# Autodesk Inventor assembly: ASY ДМФ 0100 Барабан v2.1
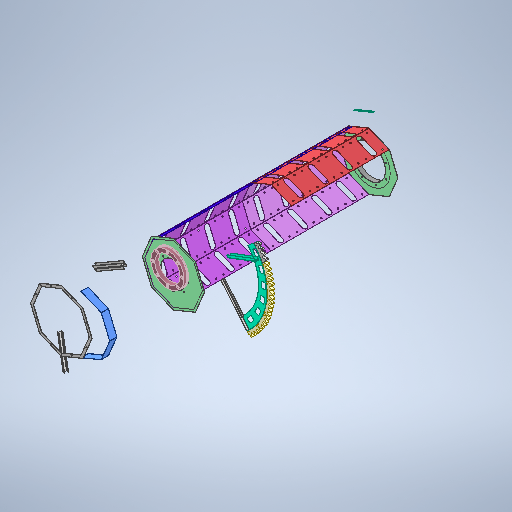
[picture p0: Inventor's stored thumbnail of the model, 512x512]
Saved by Autodesk Inventor 2026 (Build 300175000, 175)
## iProperties
Created: 2024-04-28
Part Number: ASY ДМФ 0100 Барабан v2.1
Document SubType Name: Assembly
Designer: pokla
Author: pokla
## Documents named in this file (25)
- C:\Users\pokla\Documents\Inventor\ДФО\ДМФ\DMF-Disk-Micro-Filter\Барабан v2.1\ASY ДМФ 0100 Барабан v2.1.iam
- C:\Users\pokla\Documents\Inventor\ДФО\ДМФ\DMF-Disk-Micro-Filter\Барабан v2.1\DMF 01 21 Барабан торец НОС v2.1.ipt
- C:\Users\pokla\Documents\Inventor\ДФО\ДМФ\DMF-Disk-Micro-Filter\Барабан v2.1\DMF 01 13 Барабан Лист лев брт v2.1.ipt
- C:\Users\pokla\Documents\Inventor\ДФО\ДМФ\DMF-Disk-Micro-Filter\Барабан v2.1\DMF 01 14 Барабан Лист прав брт v2.1.ipt
- C:\Users\pokla\Documents\Inventor\ДФО\ДМФ\DMF-Disk-Micro-Filter\Барабан v2.1\DMF 01 31 Барабан Опорное кольцо НОС v2.1.ipt
- C:\Users\pokla\Documents\Inventor\ДФО\ДМФ\DMF-Disk-Micro-Filter\Барабан v2.1\DMF 01 17 опора крышки v2.1.ipt
- C:\Users\pokla\Documents\Inventor\ДФО\ДМФ\DMF-Disk-Micro-Filter\Барабан v2.1\DMF 000 размеры v2.1.ipt
- C:\Users\pokla\Documents\Inventor\ДФО\ДМФ\DMF-Disk-Micro-Filter\Барабан v2.1\DMF 01 12 Барабан усилитель v2.1.ipt
- C:\Users\pokla\Documents\Inventor\ДФО\ДМФ\DMF-Disk-Micro-Filter\Барабан v2.1\ASY DMF 010 cap v2.1.iam
- C:\Users\pokla\Documents\Inventor\ДФО\ДМФ\DMF-Disk-Micro-Filter\Барабан v2.1\DMF 01 32 Барабан Опорное кольцо КОРМА v2.1.ipt
- C:\Users\pokla\Documents\Inventor\ДФО\ДМФ\DMF-Disk-Micro-Filter\Барабан v2.1\DMF 01 22 Барабан торец КОРМА v2.1.ipt
- C:\Users\pokla\Documents\Inventor\ДФО\ДМФ\DMF-Disk-Micro-Filter\Барабан v2.1\ASY DMF filter package v2.1.iam
- C:\Users\pokla\Documents\Inventor\ДФО\ДМФ\DMF-Disk-Micro-Filter\Барабан v2.1\DMF 01 21 cylinder butt end nose.ipt
- C:\Users\pokla\Documents\Inventor\ДФО\ДМФ\DMF-Disk-Micro-Filter\Барабан v2.1\DMF 2.1 01 43 Gear rim 3.ipt
- C:\Users\pokla\Documents\Inventor\ДФО\ДМФ\DMF-Disk-Micro-Filter\Барабан v2.1\DMF 2.1 01 44 Gear rim 4.ipt
- C:\Users\pokla\Documents\Inventor\ДФО\ДМФ\DMF-Disk-Micro-Filter\Барабан v2.1\DMF 2.1 01 45 Gear ring 5.ipt
- C:\Users\pokla\Documents\Inventor\ДФО\ДМФ\DMF-Disk-Micro-Filter\Барабан v2.1\DMF 2.1 01 46 Gear axis wheel 6.ipt
- C:\Users\pokla\Documents\Inventor\ДФО\ДМФ\DMF-Disk-Micro-Filter\Барабан v2.1\DMF 01 13 Барабан усилитель v2.1.ipt
- C:\Users\pokla\Documents\Inventor\ДФО\ДМФ\DMF-Disk-Micro-Filter\шестерни 06.09.2025\DMF sector big gear 2.1.ipt
- C:\Users\pokla\Documents\Inventor\ДФО\ДМФ\DMF-Disk-Micro-Filter\Барабан v2.1\DMF 01 15 drum sheet 1.ipt
- C:\Users\pokla\Documents\Inventor\ДФО\ДМФ\DMF-Disk-Micro-Filter\ДМФ 01 12 Барабан усилитель.ipt
- C:\Users\pokla\Documents\Inventor\ДФО\ДМФ\DMF-Disk-Micro-Filter\ДМФ 01 15 Барабан усилитель борта.ipt
- C:\Users\pokla\Documents\Inventor\ДФО\ДМФ\DMF-Disk-Micro-Filter\Барабан v2.1\DMF 2.1 Пластина паза маленькая.ipt
- C:\Users\pokla\Documents\Inventor\ДФО\ДМФ\DMF-Disk-Micro-Filter\Барабан v2.1\DMF 2.1 Пластина паза большая.ipt
- C:\Users\pokla\Documents\Inventor\ДФО\ДМФ\DMF-Disk-Micro-Filter\Барабан v2.1\DMF 01 11 cylinder sheet cap v2.1.ipt
## Components (43 placed, 30 different names)
1. DMF 000 размеры v2.1.ipt:1
2. DMF 01 21 Барабан торец НОС v2.1.ipt:1 — Жесткий:101, Совмещение:49
3. DMF 01 31 Барабан Опорное кольцо НОС v2.1.ipt:1
4. DMF 01 32 Барабан Опорное кольцо КОРМА v2.1.ipt:1 — Жесткий:20
5. DMF 01 22 Барабан торец КОРМА v2.1.ipt:1 — Жесткий:20, Жесткий:51, Жесткий:53, Совмещение:37, Жесткий:97, Совмещение:46
6. DMF 01 13 Барабан Лист лев брт v2.1.ipt:1 — Жесткий:51, Жесткий:98
7. DMF 01 14 Барабан Лист прав брт v2.1.ipt:1 — Жесткий:53
8. DMF 01 17 опора крышки v2.1.ipt:1 — Совмещение:37, Совмещение:46, Совмещение:47, Совмещение:48, Жесткий:112
9. DMF 01 11 cylinder sheet cap v2.1.ipt:1 — Совмещение:47, Жесткий:100
10. ASY DMF 010 cap v2.1.iam:1 [sub-assembly]
11. DMF 01 21 cylinder butt end nose.ipt:1
12. DMF 2.1 01 45 Gear ring 5.ipt:1
13. DMF 2.1 01 46 Gear axis wheel 6.ipt:1
14. DMF 2.1 01 44 Gear rim 4.ipt:1 — Жесткий:102, Жесткий:110
15. DMF 2.1 01 43 Gear rim 3.ipt:2 — Жесткий:102, Жесткий:103, Жесткий:109
16. DMF 01 15 drum sheet 1.ipt:1
17. ДМФ 01 12 Барабан усилитель.ipt:2 — Жесткий:56, Жесткий:57, Жесткий:89
18. ДМФ 01 15 Барабан усилитель борта.ipt:3 — Жесткий:56
19. ДМФ 01 15 Барабан усилитель борта.ipt:4 — Жесткий:57
20. ДМФ 01 12 Барабан усилитель:3 — Жесткий:89
21. ДМФ 01 15 Барабан усилитель борта:5
22. ДМФ 01 15 Барабан усилитель борта:6
23. DMF 01 12 Барабан усилитель v2.1.ipt:1 — Жесткий:82
24. DMF 01 13 Барабан усилитель v2.1.ipt:1 — Жесткий:82
25. DMF 01 12 Барабан усилитель v2.1.ipt:2
26. DMF 01 13 Барабан усилитель v2.1.ipt:2 — Жесткий:103
27. DMF 2.1 Пластина паза маленькая.ipt:1
28. DMF 2.1 Пластина паза большая:1 — Жесткий:110, Совмещение:49
29. ASY DMF filter package v2.1.iam:1 [sub-assembly]
30. DMF sector big gear 2.1.ipt:1 — Жесткий:104, Жесткий:109
31. ASY DMF filter package v2.1:2 [sub-assembly]
32. ASY DMF filter package v2.1:3 [sub-assembly]
33. ASY DMF filter package v2.1:4 [sub-assembly]
34. DMF 01 13 Барабан Лист лев брт v2.1:2 — Жесткий:97, Жесткий:99, Совмещение:48
35. DMF 01 13 Барабан Лист лев брт v2.1:3 — Жесткий:98
36. DMF 01 13 Барабан Лист лев брт v2.1:4 — Жесткий:99, Жесткий:101
37. DMF sector big gear 2.1:2 — Жесткий:104, Жесткий:105
38. DMF sector big gear 2.1:3 — Жесткий:105, Жесткий:106
39. DMF sector big gear 2.1:4 — Жесткий:106, Жесткий:107
40. DMF sector big gear 2.1:5 — Жесткий:107, Жесткий:108
41. DMF sector big gear 2.1:6 — Жесткий:108
42. ASY DMF filter package v2.1:5 [sub-assembly] — Жесткий:100
43. DMF 01 17 опора крышки v2.1:4 — Жесткий:112
## Relationships (34: WeldJoint 26, Mate 6, Flush 2)
- Жесткий:20 [WeldJoint]: DMF 01 32 Барабан Опорное кольцо КОРМА v2.1.ipt:1 ↔ DMF 01 22 Барабан торец КОРМА v2.1.ipt:1
- Жесткий:51 [WeldJoint]: DMF 01 22 Барабан торец КОРМА v2.1.ipt:1 ↔ DMF 01 13 Барабан Лист лев брт v2.1.ipt:1
- Жесткий:53 [WeldJoint]: DMF 01 22 Барабан торец КОРМА v2.1.ipt:1 ↔ DMF 01 14 Барабан Лист прав брт v2.1.ipt:1
- Совмещение:37 [Mate]: DMF 01 22 Барабан торец КОРМА v2.1.ipt:1 ↔ DMF 01 17 опора крышки v2.1.ipt:1
- Жесткий:56 [WeldJoint]: ДМФ 01 12 Барабан усилитель.ipt:2 ↔ ДМФ 01 15 Барабан усилитель борта.ipt:3
- Жесткий:57 [WeldJoint]: ДМФ 01 12 Барабан усилитель.ipt:2 ↔ ДМФ 01 15 Барабан усилитель борта.ipt:4
- [Mate]: DMF 01 22 Барабан торец КОРМА v2.1.ipt:1 ↔ DMF 01 11 cylinder sheet cap v2.1.ipt:1
- [Flush]: DMF 01 22 Барабан торец КОРМА v2.1.ipt:1 ↔ DMF 01 11 cylinder sheet cap v2.1.ipt:1
- [Flush]: DMF 01 22 Барабан торец КОРМА v2.1.ipt:1 ↔ DMF 01 11 cylinder sheet cap v2.1.ipt:1
- Жесткий:82 [WeldJoint]: DMF 01 12 Барабан усилитель v2.1.ipt:1 ↔ DMF 01 13 Барабан усилитель v2.1.ipt:1
- [WeldJoint]: ДМФ 01 12 Барабан усилитель:3 ↔ ДМФ 01 15 Барабан усилитель борта:5
- [WeldJoint]: ДМФ 01 12 Барабан усилитель:3 ↔ ДМФ 01 15 Барабан усилитель борта:6
- Жесткий:89 [WeldJoint]: ДМФ 01 12 Барабан усилитель.ipt:2 ↔ ДМФ 01 12 Барабан усилитель:3
- [WeldJoint]: DMF 01 11 cylinder sheet cap v2.1.ipt:1 ↔ ASY DMF filter package v2.1.iam:1
- [WeldJoint]: DMF 01 11 cylinder sheet cap v2.1.ipt:1 ↔ ASY DMF filter package v2.1:2
- Жесткий:97 [WeldJoint]: DMF 01 22 Барабан торец КОРМА v2.1.ipt:1 ↔ DMF 01 13 Барабан Лист лев брт v2.1:2
- Жесткий:98 [WeldJoint]: DMF 01 13 Барабан Лист лев брт v2.1.ipt:1 ↔ DMF 01 13 Барабан Лист лев брт v2.1:3
- Жесткий:99 [WeldJoint]: DMF 01 13 Барабан Лист лев брт v2.1:2 ↔ DMF 01 13 Барабан Лист лев брт v2.1:4
- Совмещение:46 [Mate]: DMF 01 22 Барабан торец КОРМА v2.1.ipt:1 ↔ DMF 01 17 опора крышки v2.1.ipt:1
- Совмещение:47 [Mate]: DMF 01 17 опора крышки v2.1.ipt:1 ↔ DMF 01 11 cylinder sheet cap v2.1.ipt:1
- Совмещение:48 [Mate]: DMF 01 17 опора крышки v2.1.ipt:1 ↔ DMF 01 13 Барабан Лист лев брт v2.1:2
- Жесткий:100 [WeldJoint]: DMF 01 11 cylinder sheet cap v2.1.ipt:1 ↔ ASY DMF filter package v2.1:5
- Жесткий:101 [WeldJoint]: DMF 01 21 Барабан торец НОС v2.1.ipt:1 ↔ DMF 01 13 Барабан Лист лев брт v2.1:4
- Жесткий:102 [WeldJoint]: DMF 2.1 01 44 Gear rim 4.ipt:1 ↔ DMF 2.1 01 43 Gear rim 3.ipt:2
- Жесткий:103 [WeldJoint]: DMF 2.1 01 43 Gear rim 3.ipt:2 ↔ DMF 01 13 Барабан усилитель v2.1.ipt:2
- Жесткий:104 [WeldJoint]: DMF sector big gear 2.1.ipt:1 ↔ DMF sector big gear 2.1:2
- Жесткий:105 [WeldJoint]: DMF sector big gear 2.1:2 ↔ DMF sector big gear 2.1:3
- Жесткий:106 [WeldJoint]: DMF sector big gear 2.1:3 ↔ DMF sector big gear 2.1:4
- Жесткий:107 [WeldJoint]: DMF sector big gear 2.1:4 ↔ DMF sector big gear 2.1:5
- Жесткий:108 [WeldJoint]: DMF sector big gear 2.1:5 ↔ DMF sector big gear 2.1:6
- Жесткий:109 [WeldJoint]: DMF 2.1 01 43 Gear rim 3.ipt:2 ↔ DMF sector big gear 2.1.ipt:1
- Жесткий:110 [WeldJoint]: DMF 2.1 01 44 Gear rim 4.ipt:1 ↔ DMF 2.1 Пластина паза большая:1
- Совмещение:49 [Mate] (120 mm): DMF 01 21 Барабан торец НОС v2.1.ipt:1 ↔ DMF 2.1 Пластина паза большая:1
- Жесткий:112 [WeldJoint]: DMF 01 17 опора крышки v2.1.ipt:1 ↔ DMF 01 17 опора крышки v2.1:4
## Named parameters: d460_d378 = 0 mm, d461_d379 = 0 mm
